# Autodesk Inventor assembly: Assembly waste sorting and management
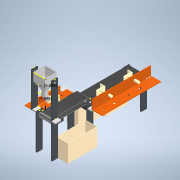
[picture p0: Inventor's stored thumbnail of the model, 180x180]
Saved by Autodesk Inventor 2021 (Build 250183000, 183)
## iProperties
Created: 2025-06-24
Part Number: Assembly waste sorting and management
Document SubType Name: Assembly
Designer: Apanzia
Author: Apanzia
## Documents named in this file (17)
- C:\Users\Apanzia\Documents\Assembly waste sorting and management.iam
- C:\Users\Apanzia\Documents\Conveyor.ipt
- C:\Users\Apanzia\Documents\Rollers.ipt
- C:\Users\Apanzia\Documents\Post.ipt
- C:\Users\Apanzia\Documents\supporter.ipt
- C:\Users\Apanzia\Documents\feeder funnel.ipt
- C:\Users\Apanzia\Documents\beam.ipt
- C:\Users\Apanzia\Documents\junction.ipt
- C:\Users\Apanzia\Documents\conveyor2.ipt
- C:\Users\Apanzia\Documents\roller2.ipt
- C:\Users\Apanzia\Documents\Part5.ipt
- C:\Users\Apanzia\Documents\bracket.ipt
- C:\Users\Apanzia\Documents\Sorter.ipt
- C:\Users\Apanzia\Documents\bracket2.ipt
- C:\Users\Apanzia\Documents\bin1.ipt
- C:\Users\Apanzia\Documents\bin2.ipt
- C:\Users\Apanzia\Documents\Part6.ipt
## Components (37 placed, 16 different names)
1. Conveyor:1 — Mate:1, Flush:1, Mate:2, Flush:2
2. Rollers:1 — Mate:2, Flush:2, Mate:3, Flush:3, Mate:4, Flush:5
3. Rollers:2 — Mate:1, Flush:1, Flush:4, Mate:5, Flush:6
4. Post:1 — Flush:4, Mate:5, Flush:6, Mate:11, Mate:13, Mate:24, Mate:33
5. Post:2 — Mate:3, Flush:3, Mate:7, Flush:8
6. Post:3 — Mate:4, Flush:5, Mate:6, Flush:7
7. Post:4 — Mate:8, Flush:9, Flush:10, Mate:9, Mate:19
8. Post:5 — Mate:10
9. supporter:1 — Mate:7, Flush:8
10. supporter:2 — Mate:6, Flush:7, Mate:8, Flush:9, Flush:10
11. feeder funnel:1 — Mate:9, Mate:10
12. beam:1 — Mate:12, Flush:12, Mate:34, Flush:15, Mate:36, Mate:37
13. junction:1 — Mate:11, Mate:12, Flush:12
14. conveyor2:1 — Mate:14, Flush:11, Mate:16, Flush:13
15. roller2:1 — Mate:16, Flush:13, Mate:17, Mate:18
16. roller2:2 — Mate:13, Mate:14, Flush:11, Mate:15
17. Part5:1 — Mate:15
18. beam:2 — Mate:17, Mate:35, Flush:16
19. beam:3 — Mate:18, Mate:25
20. bracket:1 — Mate:19, Mate:20, Mate:21, Mate:22, Flush:14, Mate:23
21. Sorter:1 — Mate:20, Mate:21
22. bracket:2 — Mate:22, Flush:14
23. bracket:3 — Mate:23
24. supporter:3 — Mate:25
25. supporter:4 — Mate:24, Mate:26, Mate:27, Mate:28
26. bracket2:1 — Mate:26, Mate:27, Mate:28, Mate:29, Mate:30, Mate:31, Mate:32
27. bracket2:2 — Mate:30, Mate:31
28. Sorter:2
29. Sorter:3 — Mate:29
30. bracket:4 — Mate:32
31. bracket:5
32. bin1:1 — Mate:33
33. bin2:1 — Mate:34, Flush:15
34. bin2:2 — Mate:35, Flush:16
35. beam:4 — Mate:38
36. Part6:1 — Mate:36
37. Part6:2 — Mate:37, Mate:38
## Relationships (54: Mate 38, Flush 16)
- Mate:1: Conveyor:1 ↔ Rollers:2
- Flush:1: Conveyor:1 ↔ Rollers:2
- Mate:2: Conveyor:1 ↔ Rollers:1
- Flush:2: Conveyor:1 ↔ Rollers:1
- Mate:3: Rollers:1 ↔ Post:2
- Flush:3: Rollers:1 ↔ Post:2
- Flush:4: Rollers:2 ↔ Post:1
- Mate:4: Rollers:1 ↔ Post:3
- Flush:5: Rollers:1 ↔ Post:3
- Mate:5: Rollers:2 ↔ Post:1
- Flush:6: Rollers:2 ↔ Post:1
- Mate:6: Post:3 ↔ supporter:2
- Flush:7: Post:3 ↔ supporter:2
- Mate:7: Post:2 ↔ supporter:1
- Flush:8: Post:2 ↔ supporter:1
- Mate:8: Post:4 ↔ supporter:2
- Flush:9: Post:4 ↔ supporter:2
- Flush:10: Post:4 ↔ supporter:2
- Mate:9: Post:4 ↔ feeder funnel:1
- Mate:10: Post:5 ↔ feeder funnel:1
- Mate:11: Post:1 ↔ junction:1
- Mate:12: beam:1 ↔ junction:1
- Mate:13: Post:1 ↔ roller2:2
- Mate:14: conveyor2:1 ↔ roller2:2
- Flush:11: conveyor2:1 ↔ roller2:2
- Flush:12: beam:1 ↔ junction:1
- Mate:15: roller2:2 ↔ Part5:1
- Mate:16: conveyor2:1 ↔ roller2:1
- Flush:13: conveyor2:1 ↔ roller2:1
- Mate:17: roller2:1 ↔ beam:2
- Mate:18: roller2:1 ↔ beam:3
- Mate:19: Post:4 ↔ bracket:1
- Mate:20: bracket:1 ↔ Sorter:1
- Mate:21: bracket:1 ↔ Sorter:1
- Mate:22: bracket:1 ↔ bracket:2
- Flush:14: bracket:1 ↔ bracket:2
- Mate:23: bracket:1 ↔ bracket:3
- Mate:24: Post:1 ↔ supporter:4
- Mate:25: beam:3 ↔ supporter:3
- Mate:26: supporter:4 ↔ bracket2:1
- Mate:27: supporter:4 ↔ bracket2:1
- Mate:28: supporter:4 ↔ bracket2:1
- Mate:29: bracket2:1 ↔ Sorter:3
- Mate:30: bracket2:1 ↔ bracket2:2
- Mate:31: bracket2:1 ↔ bracket2:2
- Mate:32: bracket2:1 ↔ bracket:4
- Mate:33: Post:1 ↔ bin1:1
- Mate:34: beam:1 ↔ bin2:1
- Flush:15: beam:1 ↔ bin2:1
- Mate:35: beam:2 ↔ bin2:2
- Flush:16: beam:2 ↔ bin2:2
- Mate:36: beam:1 ↔ Part6:1
- Mate:37: beam:1 ↔ Part6:2
- Mate:38: beam:4 ↔ Part6:2
